# Autodesk Inventor assembly: xyz_Axis_with_ball_Group
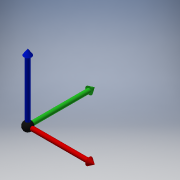
[picture p0: Inventor's stored thumbnail of the model, 180x180]
Saved by Autodesk Inventor 2018.2 (Build 222227000, 227)
## iProperties
Created: 2018-06-07
Part Number: xyz_Axis_with_ball_Group
Material: Generisch
Document SubType Name: Assembly
Designer: Nick Koch
Author: Nick Koch
## Documents named in this file (3)
- C:\Users\Nick Koch\Desktop\Lehre\FHNW\Raytracing Modell\xyz_Axis\xyz_Axis_with_ball_Group.iam
- C:\Users\Nick Koch\Desktop\Lehre\FHNW\Raytracing Modell\xyz_Axis\xyz_Axis_Ball.ipt
- C:\Users\Nick Koch\Desktop\Lehre\FHNW\Raytracing Modell\xyz_Axis\xyz_Axis_axis.ipt
## Components (4 placed, 2 different names)
1. xyz_Axis_Ball:1 — Passend:1, Passend:2, Passend:3, Passend:4, Passend:5, Passend:6
2. xyz_Axis_axis:1 — Passend:5, Passend:6
3. xyz_Axis_axis:2 — Passend:3, Passend:4
4. xyz_Axis_axis:3 — Passend:1, Passend:2
## Relationships (6: Mate 6)
- Passend:1 [Mate]: xyz_Axis_Ball:1 ↔ xyz_Axis_axis:3
- Passend:2 [Mate]: xyz_Axis_Ball:1 ↔ xyz_Axis_axis:3
- Passend:3 [Mate]: xyz_Axis_Ball:1 ↔ xyz_Axis_axis:2
- Passend:4 [Mate]: xyz_Axis_Ball:1 ↔ xyz_Axis_axis:2
- Passend:5 [Mate]: xyz_Axis_Ball:1 ↔ xyz_Axis_axis:1
- Passend:6 [Mate]: xyz_Axis_Ball:1 ↔ xyz_Axis_axis:1
